# Autodesk Inventor assembly: SeatSubassembly
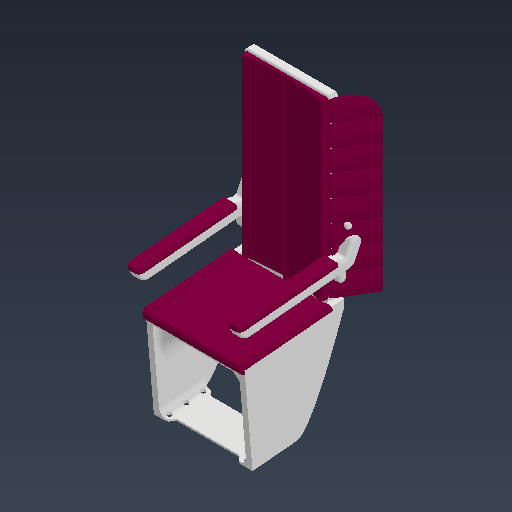
[picture p0: Inventor's stored thumbnail of the model, 512x512]
Saved by Autodesk Inventor 2021 (Build 250183000, 183)
## iProperties
Created: 2021-01-30
Part Number: SeatSubassembly
Document SubType Name: Assembly
Designer: argon
Author: argon
## Documents named in this file (11)
- C:\Users\argon\OneDrive\Documents\GrabCAD\EngOne Maroons\Seat Subassembly\SeatSubassembly.iam
- C:\Users\argon\OneDrive\Documents\GrabCAD\EngOne Maroons\Seat Subassembly\MouldedBacking.ipt
- C:\Users\argon\OneDrive\Documents\GrabCAD\EngOne Maroons\Seat Subassembly\LeftBackCushion.ipt
- C:\Users\argon\OneDrive\Documents\GrabCAD\EngOne Maroons\Seat Subassembly\RightBackCushion.ipt
- C:\Users\argon\OneDrive\Documents\GrabCAD\EngOne Maroons\Seat Subassembly\CentreBackCushion.ipt
- C:\Users\argon\OneDrive\Documents\GrabCAD\EngOne Maroons\Seat Subassembly\LeftSideCushion.ipt
- C:\Users\argon\OneDrive\Documents\GrabCAD\EngOne Maroons\Seat Subassembly\BottomSeatCushion.ipt
- C:\Users\argon\OneDrive\Documents\GrabCAD\EngOne Maroons\Seat Subassembly\RightArmRest.ipt
- C:\Users\argon\OneDrive\Documents\GrabCAD\EngOne Maroons\Seat Subassembly\ArmRestCushion.ipt
- C:\Users\argon\OneDrive\Documents\GrabCAD\EngOne Maroons\Seat Subassembly\LeftArmRest.ipt
- C:\Users\argon\OneDrive\Documents\GrabCAD\EngOne Maroons\Seat Subassembly\RightSideCushion.ipt
## Components (11 placed, 10 different names)
1. MouldedBacking:1 — Mate:1, Flush:1, Flush:2, Flush:3, Flush:5, Mate:6, Mate:7, Mate:8, Angle:2, Mate:9, Mate:14, Angle:3, Mate:15, Mate:16, Angle:4, Angle:6
2. LeftBackCushion:1 — Mate:4, Flush:3, Mate:5, Flush:4, Angle:2, Angle:5
3. RightBackCushion:1 — Mate:3, Flush:2, Mate:20, Flush:6, Angle:6, Angle:7
4. CentreBackCushion:1 — Mate:1, Mate:3, Mate:4, Flush:1, Flush:5
5. LeftSideCushion:1 — Mate:5, Flush:4, Angle:5
6. BottomSeatCushion:1 — Mate:6, Mate:7, Mate:8
7. RightArmRest:1 — Mate:9, Mate:11, Mate:12, Mate:13, Mate:14, Angle:3
8. ArmRestCushion:1 — Mate:11, Mate:12, Mate:13
9. LeftArmRest:1 — Mate:15, Mate:16, Angle:4, Mate:17, Mate:18, Mate:19
10. ArmRestCushion:2 — Mate:17, Mate:18, Mate:19
11. RightSideCushion:1 — Mate:20, Flush:6, Angle:7
## Relationships (30: Mate 18, Flush 6, Angle 6)
- Mate:1: MouldedBacking:1 ↔ CentreBackCushion:1
- Mate:3: RightBackCushion:1 ↔ CentreBackCushion:1
- Mate:4: LeftBackCushion:1 ↔ CentreBackCushion:1
- Flush:1 (-210 mm): MouldedBacking:1 ↔ CentreBackCushion:1
- Flush:2 (10 mm): MouldedBacking:1 ↔ RightBackCushion:1
- Flush:3 (10 mm): MouldedBacking:1 ↔ LeftBackCushion:1
- Mate:5: LeftBackCushion:1 ↔ LeftSideCushion:1
- Flush:4: LeftBackCushion:1 ↔ LeftSideCushion:1
- Flush:5 (10 mm): MouldedBacking:1 ↔ CentreBackCushion:1
- Mate:6: MouldedBacking:1 ↔ BottomSeatCushion:1
- Mate:7: MouldedBacking:1 ↔ BottomSeatCushion:1
- Mate:8: MouldedBacking:1 ↔ BottomSeatCushion:1
- Angle:2 (100 deg): MouldedBacking:1 ↔ LeftBackCushion:1
- Mate:9: MouldedBacking:1 ↔ RightArmRest:1
- Mate:11: RightArmRest:1 ↔ ArmRestCushion:1
- Mate:12: RightArmRest:1 ↔ ArmRestCushion:1
- Mate:13: RightArmRest:1 ↔ ArmRestCushion:1
- Mate:14: MouldedBacking:1 ↔ RightArmRest:1
- Angle:3 (-104 deg): MouldedBacking:1 ↔ RightArmRest:1
- Mate:15: MouldedBacking:1 ↔ LeftArmRest:1
- Mate:16: MouldedBacking:1 ↔ LeftArmRest:1
- Angle:4 (0 deg): MouldedBacking:1 ↔ LeftArmRest:1
- Mate:17: LeftArmRest:1 ↔ ArmRestCushion:2
- Mate:18: LeftArmRest:1 ↔ ArmRestCushion:2
- Mate:19: LeftArmRest:1 ↔ ArmRestCushion:2
- Angle:5 (180 deg): LeftBackCushion:1 ↔ LeftSideCushion:1
- Mate:20: RightBackCushion:1 ↔ RightSideCushion:1
- Flush:6: RightBackCushion:1 ↔ RightSideCushion:1
- Angle:6 (180 deg): MouldedBacking:1 ↔ RightBackCushion:1
- Angle:7 (180 deg): RightBackCushion:1 ↔ RightSideCushion:1
